# Autodesk Inventor assembly: Assembly1
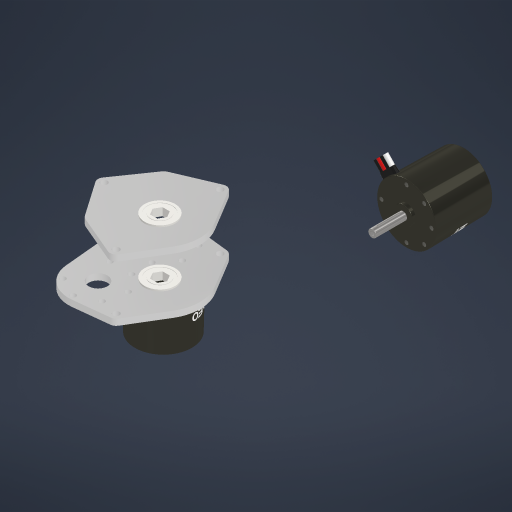
[picture p0: Inventor's stored thumbnail of the model, 512x512]
Saved by Autodesk Inventor 2024.3 (Build 283343000, 343)
## iProperties
Created: 2024-10-31
Part Number: Assembly1
Document SubType Name: Assembly
Designer: kaito
Author: kaito
## Documents named in this file (5)
- C:\Users\kaito\OneDrive\Documents\GitHub\1622-2024-Assignments\Kaito Kubota-Valme\Gearbox 2 v.2\Assembly1.iam
- C:\Users\kaito\OneDrive\Documents\GitHub\1622-2024-Assignments\Kaito Kubota-Valme\Gearbox 2 v.2\Bottom Plate.ipt
- C:\Users\kaito\OneDrive\Documents\GitHub\1622-2024-Assignments\Kaito Kubota-Valme\Gearbox 2 v.2\Part1.ipt
- C:\Users\kaito\OneDrive\Desktop\COTS Library\Motion\Bearings\COTS_WCP-0783_1.125ODHexBearing.ipt
- C:\Users\kaito\OneDrive\Desktop\Gearbox 2\REV-21-1650-V1.1.ipt
## Components (6 placed, 4 different names)
1. Bottom Plate:1 — Mate:3, Mate:4, Mate:5
2. Part1:1 — Mate:1, Mate:2, Mate:5, Mate:6, Mate:7
3. COTS_WCP-0783_1.125ODHexBearing:1 — Mate:1, Mate:2
4. COTS_WCP-0783_1.125ODHexBearing:2 — Mate:3, Mate:4
5. REV-21-1650-V1.1:1
6. REV-21-1650-V1.1:2 — Mate:6, Mate:7
## Relationships (7: Mate 7)
- Mate:1: Part1:1 ↔ COTS_WCP-0783_1.125ODHexBearing:1
- Mate:2: Part1:1 ↔ COTS_WCP-0783_1.125ODHexBearing:1
- Mate:3: Bottom Plate:1 ↔ COTS_WCP-0783_1.125ODHexBearing:2
- Mate:4: Bottom Plate:1 ↔ COTS_WCP-0783_1.125ODHexBearing:2
- Mate:5: Bottom Plate:1 ↔ Part1:1
- Mate:6: Part1:1 ↔ REV-21-1650-V1.1:2
- Mate:7: Part1:1 ↔ REV-21-1650-V1.1:2
